# Autodesk Inventor assembly: Intake 2
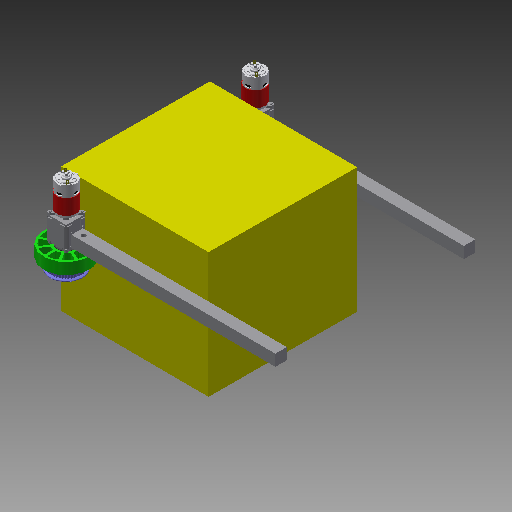
[picture p0: Inventor's stored thumbnail of the model, 512x512]
Saved by Autodesk Inventor 2018 (Build 220112000, 112)
## iProperties
Created: 2018-01-18
Part Number: Intake 2
Document SubType Name: Assembly
Designer: Apple
Author: Apple
## Documents named in this file (4)
- C:\Users\Apple\Documents\Inventor\2018 PowerUp\Cube Intake\Intake 2.iam
- C:\Users\Apple\Documents\Inventor\2018 PowerUp\2018 power cube.ipt
- C:\Users\Apple\Documents\Inventor\2018 PowerUp\Cube Intake\Sport57 with Redline and 4inc wheel.iam
- C:\Users\Apple\Documents\Inventor\2018 PowerUp\Cube Intake\Intake Arm.ipt
## Components (5 placed, 3 different names)
1. 2018 power cube:1 — Mate:6, Mate:9, Arm To Floor
2. Sport57 with Redline and 4inc wheel:1 [sub-assembly] — Flush:2, Mate:6, Mate:7, Flush:3, Flush:8
3. Intake Arm:1 — Flush:2, Mate:7, Flush:3, Flush:4, Flush:6, Arm To Floor
4. Sport57 with Redline and 4inc wheel:2 [sub-assembly] — Mate:8, Flush:5, Mate:9, Flush:8
5. Intake Arm:2 — Flush:4, Mate:8, Flush:5, Flush:6
## Relationships (11: Flush 7, Mate 4)
- Flush:2: Sport57 with Redline and 4inc wheel:1 ↔ Intake Arm:1
- Mate:6 (44.45 mm): 2018 power cube:1 ↔ Sport57 with Redline and 4inc wheel:1
- Mate:7: Sport57 with Redline and 4inc wheel:1 ↔ Intake Arm:1
- Flush:3 (-11.43 mm): Sport57 with Redline and 4inc wheel:1 ↔ Intake Arm:1
- Flush:4: Intake Arm:1 ↔ Intake Arm:2
- Mate:8: Sport57 with Redline and 4inc wheel:2 ↔ Intake Arm:2
- Flush:5 (-11.43 mm): Sport57 with Redline and 4inc wheel:2 ↔ Intake Arm:2
- Flush:6: Intake Arm:1 ↔ Intake Arm:2
- Mate:9 (44.45 mm): 2018 power cube:1 ↔ Sport57 with Redline and 4inc wheel:2
- Arm To Floor [Flush] (190.5 mm): 2018 power cube:1 ↔ Intake Arm:1
- Flush:8: Sport57 with Redline and 4inc wheel:1 ↔ Sport57 with Redline and 4inc wheel:2
## Named parameters: CompliantCompress = 6.35 mm
